# Autodesk Inventor assembly: PZT Assembly
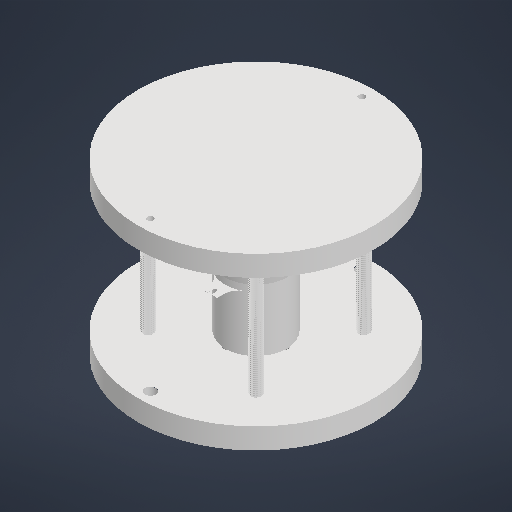
[picture p0: Inventor's stored thumbnail of the model, 512x512]
Saved by Autodesk Inventor 2025 (Build 290162000, 162)
## iProperties
Created: 2024-07-01
Part Number: PZT Assembly
Document SubType Name: Assembly
Designer: mayhe
Author: mayhe
## Documents named in this file (5)
- C:\Users\mayhe\OneDrive\Documents\GitHub\In-situ-monitoring-of-powder-bed-fusion-additive-manufacturing\system_development\Orichalcum\v0.2\Hardware_design\pzt-parts\PZT Assembly.iam
- C:\Users\mayhe\OneDrive\Documents\GitHub\In-situ-monitoring-of-powder-bed-fusion-additive-manufacturing\system_development\Orichalcum\v0.2\Hardware_design\pzt-parts\Modified Substrate Plate Top.ipt
- C:\Users\mayhe\OneDrive\Documents\GitHub\In-situ-monitoring-of-powder-bed-fusion-additive-manufacturing\system_development\Orichalcum\v0.2\Hardware_design\pzt-parts\shaker.ipt
- C:\Users\mayhe\OneDrive\Documents\GitHub\In-situ-monitoring-of-powder-bed-fusion-additive-manufacturing\system_development\Orichalcum\v0.2\Hardware_design\pzt-parts\Modified Substrate Plate Bottom.ipt
- C:\Users\mayhe\OneDrive\Documents\GitHub\In-situ-monitoring-of-powder-bed-fusion-additive-manufacturing\system_development\Orichalcum\v0.2\Hardware_design\pzt-parts\1078N29_Class 10.9 High-Strength Steel Thread.ipt
## Components (7 placed, 4 different names)
1. Modified Substrate Plate Top:1 — Rotational:1, Rotational:3, Rotational:4, Rotational:5, Rigid:1
2. shaker:1 — Rotational:1, Rotational:2
3. Modified Substrate Plate Bottom:1 — Rotational:2
4. 1078N29_Class 10.9 High-Strength Steel Thread:1 — Rotational:3
5. 1078N29_Class 10.9 High-Strength Steel Thread:2 — Rigid:1
6. 1078N29_Class 10.9 High-Strength Steel Thread:3 — Rotational:4
7. 1078N29_Class 10.9 High-Strength Steel Thread:4 — Rotational:5
## Relationships (6: RevoluteJoint 5, WeldJoint 1)
- Rotational:1 [RevoluteJoint]: Modified Substrate Plate Top:1 ↔ shaker:1
- Rotational:2 [RevoluteJoint]: shaker:1 ↔ Modified Substrate Plate Bottom:1
- Rotational:3 [RevoluteJoint]: Modified Substrate Plate Top:1 ↔ 1078N29_Class 10.9 High-Strength Steel Thread:1
- Rotational:4 [RevoluteJoint]: Modified Substrate Plate Top:1 ↔ 1078N29_Class 10.9 High-Strength Steel Thread:3
- Rotational:5 [RevoluteJoint]: Modified Substrate Plate Top:1 ↔ 1078N29_Class 10.9 High-Strength Steel Thread:4
- Rigid:1 [WeldJoint]: Modified Substrate Plate Top:1 ↔ 1078N29_Class 10.9 High-Strength Steel Thread:2
